# Autodesk Inventor assembly: 분류대_ASSEMBLY
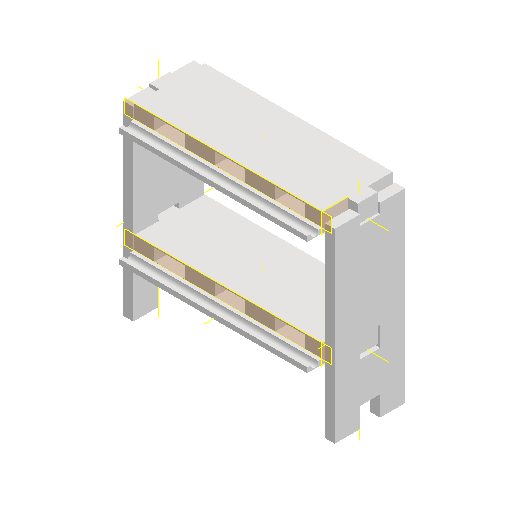
[picture p0: Inventor's stored thumbnail of the model, 512x512]
Saved by Autodesk Inventor 2027 (Build 310192000, 192)
## iProperties
Created: 2026-09-17
Part Number: 분류대_ASSEMBLY
Document SubType Name: Assembly
Designer: User
Author: User
## Documents named in this file (3)
- C:\Users\User\Desktop\4_권도영\졸업작품\INVENTOR\분류대_ASSEMBLY.iam
- C:\Users\User\Desktop\4_권도영\졸업작품\INVENTOR\분류대_ROW.ipt
- C:\Users\User\Desktop\4_권도영\졸업작품\INVENTOR\분류대_COLUMN.ipt
## Components (4 placed, 2 different names)
1. 분류대_ROW:1 — 메이트:1, 플러쉬:1, 플러쉬:2, 메이트:2
2. 분류대_ROW:2 — 메이트:1, 플러쉬:1, 플러쉬:2, 메이트:2, 메이트:3, 메이트:4
3. 분류대_COLUMN:1 — 메이트:3
4. 분류대_COLUMN:2 — 메이트:4
## Relationships (6: Mate 4, Flush 2)
- 메이트:1 [Mate] (95 mm): 분류대_ROW:1 ↔ 분류대_ROW:2
- 플러쉬:1 [Flush]: 분류대_ROW:1 ↔ 분류대_ROW:2
- 플러쉬:2 [Flush]: 분류대_ROW:1 ↔ 분류대_ROW:2
- 메이트:2 [Mate] (95 mm): 분류대_ROW:1 ↔ 분류대_ROW:2
- 메이트:3 [Mate]: 분류대_ROW:2 ↔ 분류대_COLUMN:1
- 메이트:4 [Mate]: 분류대_ROW:2 ↔ 분류대_COLUMN:2
